# Autodesk Inventor assembly: Assembly
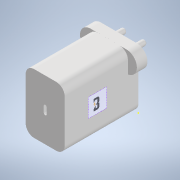
[picture p0: Inventor's stored thumbnail of the model, 180x180]
Saved by Autodesk Inventor 2022 (Build 260153000, 153)
## iProperties
Created: 2023-02-21
Part Number: Assembly
Document SubType Name: Assembly
Designer: yashm
Author: yashm
## Documents named in this file (3)
- C:\Yash\IITD\Sem 6\ELP305\ELP305_project\CAD\Assembly.iam
- C:\Yash\IITD\Sem 6\ELP305\ELP305_project\CAD\charger cover pt2.ipt
- C:\Yash\IITD\Sem 6\ELP305\ELP305_project\CAD\charger cover.ipt
## Components (2 placed, 2 different names)
1. charger cover pt2:1 — Mate:1, Mate:2, Mate:3
2. charger cover:1 — Mate:1, Mate:2, Mate:3
## Relationships (3: Mate 3)
- Mate:1: charger cover pt2:1 ↔ charger cover:1
- Mate:2: charger cover pt2:1 ↔ charger cover:1
- Mate:3: charger cover pt2:1 ↔ charger cover:1
